# Autodesk Inventor assembly: Assembly_Anglerfish_3inch_Tube_v0
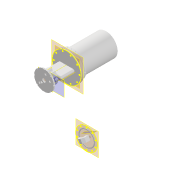
[picture p0: Inventor's stored thumbnail of the model, 180x180]
Saved by Autodesk Inventor 2022 (Build 260153000, 153)
## iProperties
Created: 2022-04-12
Part Number: Assembly_Anglerfish_3inch_Tube_v0
Document SubType Name: Assembly
Designer: Prakash Lab
Author: Prakash Lab
## Documents named in this file (13)
- C:\Users\PrakashLab\Documents\Matchboxscope\INVENTOR\Assembly_Anglerfish_3inch_Tube_v0.iam
- C:\Users\PrakashLab\Documents\Matchboxscope\INVENTOR\00_Tube_3inch.ipt
- C:\Users\PrakashLab\Documents\Matchboxscope\INVENTOR\Anglerfish_3inch_tube_endpiece.ipt
- C:\Users\PrakashLab\Documents\Matchboxscope\INVENTOR\Anglerfish_Frontwindow_3inchtube_V0.ipt
- C:\Users\PrakashLab\Documents\Matchboxscope\INVENTOR\Matchboxscope_middle2_v1.ipt
- C:\Users\PrakashLab\Documents\Matchboxscope\INVENTOR\Matchboxscope_Lightperiscope_V0.ipt
- C:\Users\PrakashLab\Documents\Matchboxscope\INVENTOR\Matchboxscope_bottom_v0.ipt
- C:\Users\PrakashLab\Documents\Matchboxscope\INVENTOR\00_ESP3-CAM.iam
- C:\Users\PrakashLab\Documents\Matchboxscope\INVENTOR\Matchboxscope_lenstube_v0.ipt
- C:\Users\PrakashLab\Documents\Matchboxscope\INVENTOR\00_Powerbank.ipt
- C:\Users\PrakashLab\Documents\Matchboxscope\INVENTOR\Anglerfish_Frontwindow_v0.ipt
- C:\Users\PrakashLab\Documents\Matchboxscope\INVENTOR\Anglerfish_rubberring_v0.ipt
- C:\Users\PrakashLab\Documents\Matchboxscope\INVENTOR\Anglerfish_3inch_tube_adapterplate_focus.ipt
## Components (13 placed, 12 different names)
1. 00_Tube_3inch:1 — Mate:6, Insert:2
2. Anglerfish_3inch_tube_endpiece:1 — Insert:2
3. Anglerfish_Frontwindow_3inchtube_V0:1
4. Matchboxscope_middle2_v1:1 — Flush:5, Flush:6
5. Matchboxscope_Lightperiscope_V0:1
6. Matchboxscope_bottom_v0:1 — Mate:6
7. 00_ESP3-CAM:1 [sub-assembly]
8. Matchboxscope_lenstube_v0:1
9. 00_Powerbank:1
10. Anglerfish_Frontwindow_v0:1
11. Anglerfish_rubberring_v0:1
12. Matchboxscope_lenstube_v0:2
13. Anglerfish_3inch_tube_adapterplate_focus:1 — Flush:5, Flush:6
## Relationships (14: Flush 6, Mate 6, Insert 2)
- [Flush]: 00_Tube_3inch:1 ↔ Anglerfish_3inch_tube_endpiece:1
- [Flush]: Anglerfish_3inch_tube_endpiece:1 ↔ Anglerfish_Frontwindow_3inchtube_V0:1
- [Flush]: Anglerfish_3inch_tube_endpiece:1 ↔ Anglerfish_Frontwindow_3inchtube_V0:1
- [Mate]: Matchboxscope_bottom_v0:1 ↔ 00_ESP3-CAM:1
- [Flush]: Matchboxscope_bottom_v0:1 ↔ 00_ESP3-CAM:1
- [Insert]: Matchboxscope_middle2_v1:1 ↔ 00_ESP3-CAM:1
- [Mate]: Matchboxscope_middle2_v1:1 ↔ Matchboxscope_bottom_v0:1
- [Mate]: Matchboxscope_bottom_v0:1 ↔ 00_Powerbank:1
- [Mate]: Matchboxscope_bottom_v0:1 ↔ 00_Powerbank:1
- [Mate] (5 mm): Matchboxscope_bottom_v0:1 ↔ 00_Powerbank:1
- Mate:6: 00_Tube_3inch:1 ↔ Matchboxscope_bottom_v0:1
- Insert:2: 00_Tube_3inch:1 ↔ Anglerfish_3inch_tube_endpiece:1
- Flush:5: Matchboxscope_middle2_v1:1 ↔ Anglerfish_3inch_tube_adapterplate_focus:1
- Flush:6: Matchboxscope_middle2_v1:1 ↔ Anglerfish_3inch_tube_adapterplate_focus:1
## Named parameters: d3_d8 = 0 mm
